# Autodesk Inventor assembly: Degree of freedom model
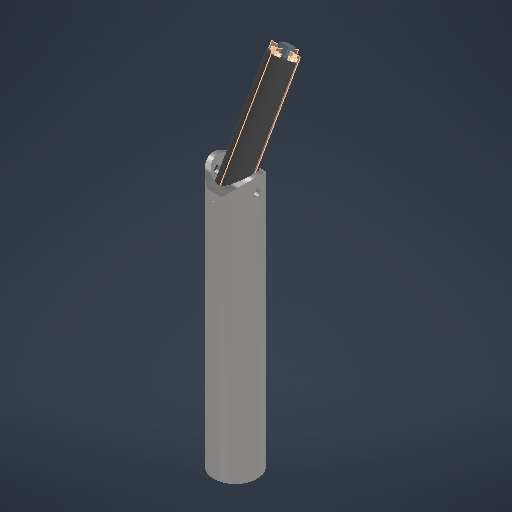
[picture p0: Inventor's stored thumbnail of the model, 512x512]
Saved by Autodesk Inventor 2026.2 (Build 302298010, 298A)
## iProperties
Created: 2026-04-01
Part Number: Degree of freedom model
Document SubType Name: Assembly
Designer: piete
Author: piete
## Documents named in this file (5)
- C:\Users\piete\Desktop\Skripsie\Documents\Concept Designs\Concept 3 1 Degree of Freedom\Degree of freedom model.iam
- C:\Users\piete\Desktop\Skripsie\Documents\Concept Designs\Concept 3 1 Degree of Freedom\Steel rod.ipt
- C:\Users\piete\Desktop\Skripsie\Documents\Concept Designs\Concept 3 1 Degree of Freedom\Camera Encasing.ipt
- C:\Users\piete\Desktop\Skripsie\Documents\Concept Designs\Camera sensor.ipt
- C:\Users\piete\Desktop\Skripsie\Documents\Concept Designs\Small light.ipt
## Components (7 placed, 4 different names)
1. Steel rod:1 — Angle:1, Mate:6, Flush:1
2. Camera Encasing:1 — Mate:3, Mate:4, Mate:5, Angle:1, Mate:6, Flush:1, Mate:7, Mate:9, Mate:10, Mate:11, Mate:12, Mate:13, Mate:14, Mate:15, Mate:16, Mate:17, Flush:2, Mate:18
3. Camera sensor:1 — Mate:3, Mate:4, Mate:5
4. Small light:1 — Mate:10, Mate:11, Mate:16
5. Small light:2 — Mate:9, Mate:12, Mate:18
6. Small light:3 — Mate:7, Mate:13, Flush:2
7. Small light:4 — Mate:14, Mate:15, Mate:17
## Relationships (18: Mate 15, Flush 2, Angle 1)
- Mate:3: Camera Encasing:1 ↔ Camera sensor:1
- Mate:4 (-1 mm): Camera Encasing:1 ↔ Camera sensor:1
- Mate:5 (-1 mm): Camera Encasing:1 ↔ Camera sensor:1
- Angle:1 (0 deg): Steel rod:1 ↔ Camera Encasing:1
- Mate:6: Steel rod:1 ↔ Camera Encasing:1
- Flush:1: Steel rod:1 ↔ Camera Encasing:1
- Mate:7: Camera Encasing:1 ↔ Small light:3
- Mate:9: Camera Encasing:1 ↔ Small light:2
- Mate:10: Camera Encasing:1 ↔ Small light:1
- Mate:11: Camera Encasing:1 ↔ Small light:1
- Mate:12: Camera Encasing:1 ↔ Small light:2
- Mate:13: Camera Encasing:1 ↔ Small light:3
- Mate:14: Camera Encasing:1 ↔ Small light:4
- Mate:15: Camera Encasing:1 ↔ Small light:4
- Mate:16 (2 mm): Camera Encasing:1 ↔ Small light:1
- Mate:17 (-2 mm): Camera Encasing:1 ↔ Small light:4
- Flush:2 (-2 mm): Camera Encasing:1 ↔ Small light:3
- Mate:18 (-2 mm): Camera Encasing:1 ↔ Small light:2
